# Autodesk Inventor assembly: blob_all
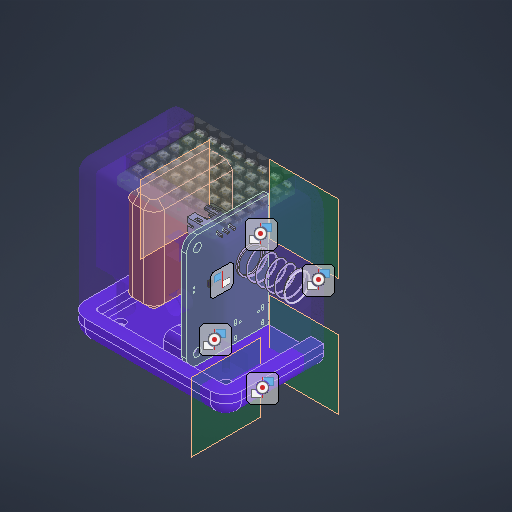
[picture p0: Inventor's stored thumbnail of the model, 512x512]
Saved by Autodesk Inventor 2026.1 (Build 301233000, 233)
## iProperties
Created: 2025-06-28
Part Number: blob_all
Document SubType Name: Assembly
Designer: micyg
Author: micyg
## Documents named in this file (7)
- C:\Users\micyg\Projects\virtual_pet\VirtualBlob\Mechanical\blob_all.iam
- C:\Users\micyg\Projects\virtual_pet\VirtualBlob\Mechanical\case1.ipt
- C:\Users\micyg\Projects\virtual_pet\VirtualBlob\Mechanical\case2.ipt
- C:\Users\micyg\Projects\virtual_pet\VirtualBlob\Mechanical\battery.ipt
- C:\Users\micyg\Projects\virtual_pet\VirtualBlob\Mechanical\matrix\matrix_V2.iam
- C:\Users\micyg\Projects\virtual_pet\VirtualBlob\Mechanical\boards\MainBoard\mainboard_0_4_0\VirtualBlob_MainBoard_0.4.0\VirtualBlob_MainBoard_0.4.0.iam
- C:\Users\micyg\Projects\virtual_pet\VirtualBlob\Mechanical\touchSpring.ipt
## Components (6 placed, 6 different names)
1. case1:1 — Zestawiające:1, Zestawiające:3, Zestawiające:5, Zestawiające:7, Zestawiające:8, Zestawiające:9, Zestawiające:17, Zestawiające:18, Zestawiające:19, Zestawiające:20
2. case2:1 — Zestawiające:3, Zestawiające:9, Zestawiające:10, Zestawiające:11, Zestawiające:12, Zestawiające:20
3. battery:1 — Zestawiające:1, Zestawiające:17, Zestawiające:18, Zestawiające:19
4. matrix_V2:1 [sub-assembly] — Zestawiające:5, Zestawiające:7, Zestawiające:8
5. VirtualBlob_MainBoard_0.4.0:1 [sub-assembly] — Zestawiające:10, Zestawiające:11, Zestawiające:12, Zestawiające:14, Zestawiające:15, Zestawiające:16
6. touchSpring:1 — Zestawiające:14, Zestawiające:15, Zestawiające:16
## Relationships (16: Mate 16)
- Zestawiające:1 [Mate] (3 mm): case1:1 ↔ battery:1
- Zestawiające:3 [Mate]: case1:1 ↔ case2:1
- Zestawiające:5 [Mate]: case1:1 ↔ matrix_V2:1
- Zestawiające:7 [Mate] (0.25 mm): case1:1 ↔ matrix_V2:1
- Zestawiające:8 [Mate] (0.25 mm): case1:1 ↔ matrix_V2:1
- Zestawiające:9 [Mate]: case1:1 ↔ case2:1
- Zestawiające:10 [Mate]: case2:1 ↔ VirtualBlob_MainBoard_0.4.0:1
- Zestawiające:11 [Mate]: case2:1 ↔ VirtualBlob_MainBoard_0.4.0:1
- Zestawiające:12 [Mate]: case2:1 ↔ VirtualBlob_MainBoard_0.4.0:1
- Zestawiające:14 [Mate]: VirtualBlob_MainBoard_0.4.0:1 ↔ touchSpring:1
- Zestawiające:15 [Mate]: VirtualBlob_MainBoard_0.4.0:1 ↔ touchSpring:1
- Zestawiające:16 [Mate]: VirtualBlob_MainBoard_0.4.0:1 ↔ touchSpring:1
- Zestawiające:17 [Mate]: case1:1 ↔ battery:1
- Zestawiające:18 [Mate]: case1:1 ↔ battery:1
- Zestawiające:19 [Mate]: case1:1 ↔ battery:1
- Zestawiające:20 [Mate]: case1:1 ↔ case2:1
